# Autodesk Inventor assembly: assembly
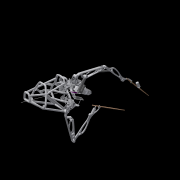
[picture p0: Inventor's stored thumbnail of the model, 180x180]
Saved by Autodesk Inventor 2020 (Build 240168000, 168)
## iProperties
Created: 2020-03-24
Part Number: assembly
Document SubType Name: Assembly
Designer: valer
Author: valer
## Documents named in this file (21)
- C:\Users\valer\Desktop\drummingrobot\src\Robot.iam
- C:\Users\valer\Desktop\drummingrobot\src\Chest.ipt
- C:\Users\valer\Desktop\drummingrobot\src\HeadScaled.ipt
- C:\Users\valer\Desktop\drummingrobot\src\UpperArmServoDynamixelXM430-W350-T.ipt
- C:\Users\valer\Desktop\drummingrobot\src\UpperArm.ipt
- C:\Users\valer\Desktop\drummingrobot\src\UpperArmBracket.ipt
- C:\Users\valer\Desktop\drummingrobot\src\UpperArmMount.ipt
- C:\Users\valer\Desktop\drummingrobot\src\external\ShoulderConnectingRod.ipt
- C:\Users\valer\Desktop\drummingrobot\src\Forearm.ipt
- C:\Users\valer\Desktop\drummingrobot\src\external\Drumstick.ipt
- C:\Users\valer\Desktop\drummingrobot\src\external\ShaftCollar1-2.ipt
- C:\Users\valer\Desktop\drummingrobot\src\external\RodEndFixed.ipt
- C:\Users\valer\Desktop\drummingrobot\src\ShoulderBracket.ipt
- C:\Users\valer\Desktop\drummingrobot\src\ChestShoulderBracket.ipt
- C:\Users\valer\Desktop\drummingrobot\src\ChestShoulderBracketMirror.ipt
- C:\Users\valer\Desktop\drummingrobot\src\external\PullSolenoid.ipt
- C:\Users\valer\Desktop\drummingrobot\src\external\PushSolenoid.ipt
- C:\Users\valer\Desktop\drummingrobot\src\external\UpperArmLinearActuatorBody.ipt
- C:\Users\valer\Desktop\drummingrobot\src\external\UpperArmLinearActuatorShaft.ipt
- C:\Users\valer\Desktop\drummingrobot\src\external\ForearmLinearActuatorBody.ipt
- C:\Users\valer\Desktop\drummingrobot\src\external\ForearmLinearActuatorShaft.ipt
## Components (56 placed, 19 different names)
1. Chest:1 — Angle:1, Angle:6, Mate:117, Mate:118, Mate:119, Mate:120, Mate:121, Mate:122, Mate:130, Mate:131, Mate:132, Mate:133, Mate:134, Mate:157
2. HeadScaled:1 — Angle:6
3. UpperArmServoDynamixelXM430-W350-T:1 — Angle:1, Mate:10, Mate:11, Mate:116, Angle:7, Mate:164
4. UpperArm:1 — Mate:3, Mate:4, Mate:5, Mate:61, Mate:64, Mate:185, Mate:189
5. UpperArmBracket:1 — Mate:3, Mate:6, Mate:8, Mate:25, Angle:8
6. UpperArmMount:1 — Mate:6, Mate:7, Mate:8, Mate:10, Mate:11, Mate:25, Mate:78, Mate:186
7. UpperArmBracket:2 — Mate:4, Mate:5, Mate:7, Mate:78
8. ChestConnectingRod:1 — Mate:88, Mate:89, Mate:105
9. ChestConnectingRod:2 — Mate:86, Mate:87, Mate:104
10. ChestConnectingRod:3 — Mate:84, Mate:85, Mate:98
11. ChestConnectingRod:4 — Mate:82, Mate:83, Mate:97
12. Forearm:1 — Mate:61, Mate:64, Mate:80, Mate:190
13. Drumstick:1 — Mate:79, Flush:3
14. ShaftCollar1/2:1 — Mate:79, Flush:3, Mate:80
15. RodEnd1/4-1/4-1:1 — Mate:82, Mate:115
16. RodEnd1/4-1/4-1:2 — Mate:83, Mate:97, Mate:123, Mate:125
17. RodEnd1/4-1/4-1:3 — Mate:84, Mate:114
18. RodEnd1/4-1/4-1:4 — Mate:85, Mate:98, Mate:124, Mate:142
19. RodEnd1/4-1/4-1:5 — Mate:86, Mate:110
20. RodEnd1/4-1/4-1:6 — Mate:87, Mate:104, Mate:126, Mate:129
21. RodEnd1/4-1/4-1:7 — Mate:88, Mate:109
22. RodEnd1/4-1/4-1:8 — Mate:89, Mate:105, Mate:127, Mate:128
23. ShoulderBracket:2 — Mate:109, Mate:110, Flush:6, Flush:7, Mate:116, Angle:7, Flush:9, Mate:164
24. ShoulderBracket:3 — Flush:6, Mate:114, Mate:115, Flush:7, Flush:8
25. ChestShoulderBracket:1 — Mate:120, Mate:121, Mate:122, Mate:123, Mate:124, Flush:8, Mate:125, Mate:142
26. ChestShoulderBracketMirror:1 — Mate:117, Mate:118, Mate:119, Mate:126, Mate:127, Flush:9, Mate:128, Mate:129
27. ChestShoulderBracket:2 — Mate:130, Mate:131, Mate:156, Mate:157, Mate:160, Mate:161, Mate:162
28. ShoulderBracket:4 — Mate:144, Mate:145, Mate:147
29. ShoulderBracket:5 — Mate:158, Mate:159, Mate:163, Mate:179, Mate:180
30. ChestShoulderBracketMirror:2 — Mate:132, Mate:133, Mate:134, Mate:141, Mate:146, Mate:148, Mate:149
31. ChestConnectingRod:5
32. ChestConnectingRod:6
33. RodEnd1/4-1/4-1:9 — Mate:144, Mate:145
34. RodEnd1/4-1/4-1:10 — Mate:148, Mate:149
35. RodEnd1/4-1/4-1:11 — Mate:147
36. RodEnd1/4-1/4-1:12 — Mate:141, Mate:146
37. ChestConnectingRod:7
38. ChestConnectingRod:8
39. RodEnd1/4-1/4-1:13 — Mate:163
40. RodEnd1/4-1/4-1:14 — Mate:161, Mate:162
41. RodEnd1/4-1/4-1:15 — Mate:158, Mate:159
42. RodEnd1/4-1/4-1:16 — Mate:156, Mate:160
43. UpperArmServoDynamixelXM430-W350-T:2 — Mate:179, Mate:180
44. UpperArm:2
45. UpperArmBracket:3
46. UpperArmMount:2
47. UpperArmBracket:4
48. Forearm:2
49. Drumstick:2 — Mate:181
50. ShaftCollar1/2:2 — Mate:181
51. PullSolenoid:1
52. PushSolenoid:1
53. FA-35-S-12-1:1 — Mate:182, Mate:183, Angle:8, Mate:186
54. FA-35-S-12-1:2 — Mate:182, Mate:183, Mate:185
55. ForearmLinearActuatorBody:1 — Mate:187, Mate:188, Mate:189
56. ForearmLinearActuatorShaft:1 — Mate:187, Mate:188, Mate:190
## Relationships (114: Mate 102, Flush 8, Angle 4)
- Angle:1 (0 deg): Chest:1 ↔ UpperArmServoDynamixelXM430-W350-T:1
- Mate:3: UpperArm:1 ↔ UpperArmBracket:1
- Mate:4: UpperArm:1 ↔ UpperArmBracket:2
- Mate:5: UpperArm:1 ↔ UpperArmBracket:2
- Mate:6: UpperArmBracket:1 ↔ UpperArmMount:1
- Mate:7: UpperArmMount:1 ↔ UpperArmBracket:2
- Mate:8: UpperArmBracket:1 ↔ UpperArmMount:1
- Mate:10: UpperArmServoDynamixelXM430-W350-T:1 ↔ UpperArmMount:1
- Mate:11: UpperArmServoDynamixelXM430-W350-T:1 ↔ UpperArmMount:1
- Mate:25 (12.7 mm): UpperArmBracket:1 ↔ UpperArmMount:1
- Angle:6 (0 deg): Chest:1 ↔ HeadScaled:1
- Mate:61: UpperArm:1 ↔ Forearm:1
- Mate:64: UpperArm:1 ↔ Forearm:1
- Mate:78: UpperArmMount:1 ↔ UpperArmBracket:2
- Mate:79: Drumstick:1 ↔ ShaftCollar1/2:1
- Flush:3 (304.8 mm): Drumstick:1 ↔ ShaftCollar1/2:1
- Mate:80: Forearm:1 ↔ ShaftCollar1/2:1
- Mate:82: ChestConnectingRod:4 ↔ RodEnd1/4-1/4-1:1
- Mate:83: ChestConnectingRod:4 ↔ RodEnd1/4-1/4-1:2
- Mate:84: ChestConnectingRod:3 ↔ RodEnd1/4-1/4-1:3
- Mate:85: ChestConnectingRod:3 ↔ RodEnd1/4-1/4-1:4
- Mate:86: ChestConnectingRod:2 ↔ RodEnd1/4-1/4-1:5
- Mate:87: ChestConnectingRod:2 ↔ RodEnd1/4-1/4-1:6
- Mate:88: ChestConnectingRod:1 ↔ RodEnd1/4-1/4-1:7
- Mate:89: ChestConnectingRod:1 ↔ RodEnd1/4-1/4-1:8
- Mate:97 (-25.4 mm): ChestConnectingRod:4 ↔ RodEnd1/4-1/4-1:2
- Mate:98 (-25.4 mm): ChestConnectingRod:3 ↔ RodEnd1/4-1/4-1:4
- Mate:104 (-25.4 mm): ChestConnectingRod:2 ↔ RodEnd1/4-1/4-1:6
- Mate:105 (-25.4 mm): ChestConnectingRod:1 ↔ RodEnd1/4-1/4-1:8
- Mate:109: RodEnd1/4-1/4-1:7 ↔ ShoulderBracket:2
- Mate:110: RodEnd1/4-1/4-1:5 ↔ ShoulderBracket:2
- Flush:6: ShoulderBracket:2 ↔ ShoulderBracket:3
- Mate:114: RodEnd1/4-1/4-1:3 ↔ ShoulderBracket:3
- Mate:115: RodEnd1/4-1/4-1:1 ↔ ShoulderBracket:3
- Flush:7: ShoulderBracket:2 ↔ ShoulderBracket:3
- Mate:116: UpperArmServoDynamixelXM430-W350-T:1 ↔ ShoulderBracket:2
- Angle:7 (0 deg): UpperArmServoDynamixelXM430-W350-T:1 ↔ ShoulderBracket:2
- Mate:117: Chest:1 ↔ ChestShoulderBracketMirror:1
- Mate:118: Chest:1 ↔ ChestShoulderBracketMirror:1
- Mate:119: Chest:1 ↔ ChestShoulderBracketMirror:1
- Mate:120: Chest:1 ↔ ChestShoulderBracket:1
- Mate:121: Chest:1 ↔ ChestShoulderBracket:1
- Mate:122: Chest:1 ↔ ChestShoulderBracket:1
- Mate:123: RodEnd1/4-1/4-1:2 ↔ ChestShoulderBracket:1
- Mate:124: RodEnd1/4-1/4-1:4 ↔ ChestShoulderBracket:1
- Flush:8: ShoulderBracket:3 ↔ ChestShoulderBracket:1
- Mate:125: RodEnd1/4-1/4-1:2 ↔ ChestShoulderBracket:1
- Mate:126: RodEnd1/4-1/4-1:6 ↔ ChestShoulderBracketMirror:1
- Mate:127: RodEnd1/4-1/4-1:8 ↔ ChestShoulderBracketMirror:1
- Flush:9: ShoulderBracket:2 ↔ ChestShoulderBracketMirror:1
- Mate:128: RodEnd1/4-1/4-1:8 ↔ ChestShoulderBracketMirror:1
- Mate:129: RodEnd1/4-1/4-1:6 ↔ ChestShoulderBracketMirror:1
- Mate:130: Chest:1 ↔ ChestShoulderBracket:2
- Mate:131: Chest:1 ↔ ChestShoulderBracket:2
- [Flush]: ShoulderBracket:4 ↔ ShoulderBracket:5
- [Flush]: ShoulderBracket:4 ↔ ShoulderBracket:5
- Mate:132: Chest:1 ↔ ChestShoulderBracketMirror:2
- Mate:133: Chest:1 ↔ ChestShoulderBracketMirror:2
- Mate:134: Chest:1 ↔ ChestShoulderBracketMirror:2
- [Mate]: ChestConnectingRod:6 ↔ RodEnd1/4-1/4-1:9
- [Mate]: ChestConnectingRod:6 ↔ RodEnd1/4-1/4-1:10
- [Mate]: ChestConnectingRod:5 ↔ RodEnd1/4-1/4-1:11
- [Mate]: ChestConnectingRod:5 ↔ RodEnd1/4-1/4-1:12
- [Mate] (-25.4 mm): ChestConnectingRod:6 ↔ RodEnd1/4-1/4-1:10
- [Mate] (-25.4 mm): ChestConnectingRod:5 ↔ RodEnd1/4-1/4-1:12
- Mate:141: ChestShoulderBracketMirror:2 ↔ RodEnd1/4-1/4-1:12
- Mate:142: RodEnd1/4-1/4-1:4 ↔ ChestShoulderBracket:1
- Mate:144: ShoulderBracket:4 ↔ RodEnd1/4-1/4-1:9
- Mate:145: ShoulderBracket:4 ↔ RodEnd1/4-1/4-1:9
- Mate:146: ChestShoulderBracketMirror:2 ↔ RodEnd1/4-1/4-1:12
- Mate:147: ShoulderBracket:4 ↔ RodEnd1/4-1/4-1:11
- Mate:148: ChestShoulderBracketMirror:2 ↔ RodEnd1/4-1/4-1:10
- Mate:149: ChestShoulderBracketMirror:2 ↔ RodEnd1/4-1/4-1:10
- [Mate]: ChestConnectingRod:8 ↔ RodEnd1/4-1/4-1:13
- [Mate]: ChestConnectingRod:8 ↔ RodEnd1/4-1/4-1:14
- [Mate]: ChestConnectingRod:7 ↔ RodEnd1/4-1/4-1:15
- [Mate]: ChestConnectingRod:7 ↔ RodEnd1/4-1/4-1:16
- [Mate] (-25.4 mm): ChestConnectingRod:8 ↔ RodEnd1/4-1/4-1:14
- [Mate] (-25.4 mm): ChestConnectingRod:7 ↔ RodEnd1/4-1/4-1:16
- Mate:156: ChestShoulderBracket:2 ↔ RodEnd1/4-1/4-1:16
- Mate:157: Chest:1 ↔ ChestShoulderBracket:2
- Mate:158: ShoulderBracket:5 ↔ RodEnd1/4-1/4-1:15
- Mate:159: ShoulderBracket:5 ↔ RodEnd1/4-1/4-1:15
- Mate:160: ChestShoulderBracket:2 ↔ RodEnd1/4-1/4-1:16
- Mate:161: ChestShoulderBracket:2 ↔ RodEnd1/4-1/4-1:14
- Mate:162: ChestShoulderBracket:2 ↔ RodEnd1/4-1/4-1:14
- Mate:163: ShoulderBracket:5 ↔ RodEnd1/4-1/4-1:13
- Mate:164 (12.7 mm): UpperArmServoDynamixelXM430-W350-T:1 ↔ ShoulderBracket:2
- [Mate]: UpperArm:2 ↔ UpperArmBracket:3
- [Mate]: UpperArm:2 ↔ UpperArmBracket:4
- [Mate]: UpperArm:2 ↔ UpperArmBracket:4
- [Mate]: UpperArmBracket:3 ↔ UpperArmMount:2
- [Mate]: UpperArmMount:2 ↔ UpperArmBracket:4
- [Mate]: UpperArmBracket:3 ↔ UpperArmMount:2
- [Mate]: UpperArmServoDynamixelXM430-W350-T:2 ↔ UpperArmMount:2
- [Mate]: UpperArmServoDynamixelXM430-W350-T:2 ↔ UpperArmMount:2
- [Mate] (12.7 mm): UpperArmBracket:3 ↔ UpperArmMount:2
- [Mate]: UpperArm:2 ↔ Forearm:2
- [Mate]: UpperArm:2 ↔ Forearm:2
- [Mate]: UpperArmMount:2 ↔ UpperArmBracket:4
- [Flush] (304.8 mm): Drumstick:2 ↔ ShaftCollar1/2:2
- [Mate]: Forearm:2 ↔ ShaftCollar1/2:2
- Mate:179 (12.7 mm): ShoulderBracket:5 ↔ UpperArmServoDynamixelXM430-W350-T:2
- Mate:180: ShoulderBracket:5 ↔ UpperArmServoDynamixelXM430-W350-T:2
- Mate:181: Drumstick:2 ↔ ShaftCollar1/2:2
- Mate:182: FA-35-S-12-1:1 ↔ FA-35-S-12-1:2
- Mate:183: FA-35-S-12-1:1 ↔ FA-35-S-12-1:2
- Mate:185: UpperArm:1 ↔ FA-35-S-12-1:2
- Angle:8 (0 deg): UpperArmBracket:1 ↔ FA-35-S-12-1:1
- Mate:186: UpperArmMount:1 ↔ FA-35-S-12-1:1
- Mate:187: ForearmLinearActuatorBody:1 ↔ ForearmLinearActuatorShaft:1
- Mate:188 (53.8226 mm): ForearmLinearActuatorBody:1 ↔ ForearmLinearActuatorShaft:1
- Mate:189: UpperArm:1 ↔ ForearmLinearActuatorBody:1
- Mate:190: Forearm:1 ↔ ForearmLinearActuatorShaft:1
## Named parameters: d236_d209 = 0 mm, d237_d212 = 0 mm, d244_d149 = 0 mm, d245_d150 = 0 mm, d246_d151 = 0 mm, d247_d152 = 0 mm, d248_d197 = -25.4 mm, d249_d198 = -25.4 mm, d259_d145 = 0 mm, d260_d146 = 0 mm, d261_d147 = 0 mm, d262_d148 = 0 mm, d263_d190 = -25.4 mm, d264_d191 = -25.4 mm, d274_d140 = 0 mm, d276_d142 = 304.8 mm, d277_d143 = 0 mm, d278_d53 = 0 mm, d279_d54 = 0 mm, d280_d55 = 0 mm, d281_d56 = 0 mm, d282_d57 = 0 mm, d283_d58 = 0 mm, d284_d60 = 0 mm, d285_d61 = 0 mm, d286_d80 = 12.7 mm, d287_d121 = 0 mm, d288_d126 = 0 mm
